# Autodesk Inventor assembly: Assembly
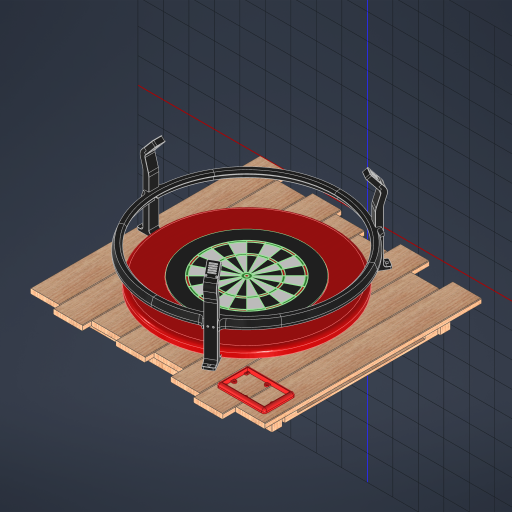
[picture p0: Inventor's stored thumbnail of the model, 512x512]
Saved by Autodesk Inventor 2023.2 (Build 272271030, 271C)
## iProperties
Created: 2023-02-18
Part Number: Assembly
Document SubType Name: Assembly
Designer: Stefan
Author: Stefan
## Documents named in this file (8)
- C:\Users\Stefan\OneDrive\Projekte\Autodarts\Inventor\Assembly.iam
- C:\Users\Stefan\OneDrive\Projekte\Autodarts\Inventor\LED-Ring_Camera-Arm.iam
- C:\Users\Stefan\OneDrive\Projekte\Autodarts\Inventor\LED-Ring_Element_v2.ipt
- C:\Users\Stefan\OneDrive\Projekte\Autodarts\Inventor\Dartboard.ipt
- C:\Users\Stefan\OneDrive\Projekte\Autodarts\Inventor\Backboard.ipt
- C:\Users\Stefan\OneDrive\Projekte\Autodarts\Inventor\Surround.ipt
- C:\Users\Stefan\OneDrive\Projekte\Autodarts\Inventor\Drawer.ipt
- C:\Users\Stefan\OneDrive\Projekte\Autodarts\Inventor\Display_Bevel.ipt
## Components (11 placed, 7 different names)
1. LED-Ring_Element_v2:1 — Passend:3, Passend:4, Passend:5
2. LED-Ring_Element_v2:2 — Passend:1, Passend:2, Passend:6
3. LED-Ring_Element_v2:3 — Passend:7, Passend:8, Passend:9, Passend:10, Passend:11, Passend:12
4. Dartboard:1 — Passend:13, Fluchtend:2
5. Surround:1 — Passend:13, Fluchtend:2
6. Backboard:1 — Fluchtend:1, Passend:15, Passend:18, Passend:19
7. Drawer:1 — Passend:15, Passend:18
8. Display_Bevel:1 — Passend:19
9. LED-Ring_Camera-Arm:1 [sub-assembly] — Passend:1, Passend:2, Passend:3, Passend:4, Passend:5, Passend:6
10. LED-Ring_Camera-Arm:2 [sub-assembly] — Passend:9, Passend:10, Passend:11
11. LED-Ring_Camera-Arm:3 [sub-assembly] — Passend:7, Passend:8, Passend:12
## Component patterns: (3 elements, first: LED-Ring_Camera-Arm:1)
## Relationships (18: Mate 16, Flush 2)
- Passend:1 [Mate]: LED-Ring_Element_v2:2 ↔ LED-Ring_Camera-Arm:1
- Passend:2 [Mate]: LED-Ring_Element_v2:2 ↔ LED-Ring_Camera-Arm:1
- Passend:3 [Mate]: LED-Ring_Element_v2:1 ↔ LED-Ring_Camera-Arm:1
- Passend:4 [Mate]: LED-Ring_Element_v2:1 ↔ LED-Ring_Camera-Arm:1
- Passend:5 [Mate]: LED-Ring_Element_v2:1 ↔ LED-Ring_Camera-Arm:1
- Passend:6 [Mate]: LED-Ring_Element_v2:2 ↔ LED-Ring_Camera-Arm:1
- Passend:7 [Mate]: LED-Ring_Element_v2:3 ↔ LED-Ring_Camera-Arm:3
- Passend:8 [Mate]: LED-Ring_Element_v2:3 ↔ LED-Ring_Camera-Arm:3
- Passend:9 [Mate]: LED-Ring_Element_v2:3 ↔ LED-Ring_Camera-Arm:2
- Passend:10 [Mate]: LED-Ring_Element_v2:3 ↔ LED-Ring_Camera-Arm:2
- Passend:11 [Mate]: LED-Ring_Element_v2:3 ↔ LED-Ring_Camera-Arm:2
- Passend:12 [Mate]: LED-Ring_Element_v2:3 ↔ LED-Ring_Camera-Arm:3
- Fluchtend:1 [Flush]: Backboard:1
- Passend:13 [Mate]: Dartboard:1 ↔ Surround:1
- Fluchtend:2 [Flush]: Dartboard:1 ↔ Surround:1
- Passend:15 [Mate] (12.5 mm): Backboard:1 ↔ Drawer:1
- Passend:18 [Mate] (10 mm): Backboard:1 ↔ Drawer:1
- Passend:19 [Mate]: Backboard:1 ↔ Display_Bevel:1
